# Autodesk Inventor assembly: LamparaSe
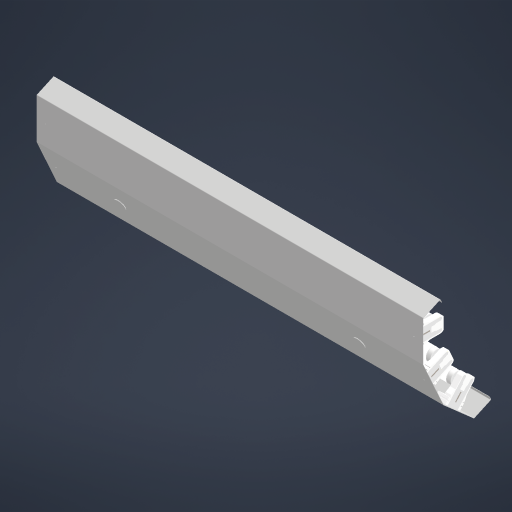
[picture p0: Inventor's stored thumbnail of the model, 512x512]
Saved by Autodesk Inventor 2024 (Build 280153000, 153)
## iProperties
Created: 2023-04-23
Part Number: LamparaSe
Document SubType Name: Assembly
Designer: javie
Author: javie
## Documents named in this file (3)
- C:\Users\javie\Downloads\LamparaSe.iam
- C:\Users\javie\Downloads\Carcasa.ipt
- C:\Users\javie\Downloads\Lampara_Secado.ipt
## Components (4 placed, 2 different names)
1. Carcasa:1 — Insertar:1, Insertar:2, Insertar:3
2. Lampara_Secado:1 — Insertar:1
3. Lampara_Secado:2 — Insertar:3
4. Lampara_Secado:3 — Insertar:2
## Relationships (3: Insert 3)
- Insertar:1: Carcasa:1 ↔ Lampara_Secado:1
- Insertar:2: Carcasa:1 ↔ Lampara_Secado:3
- Insertar:3: Carcasa:1 ↔ Lampara_Secado:2
